# Autodesk Inventor assembly: Computer Case
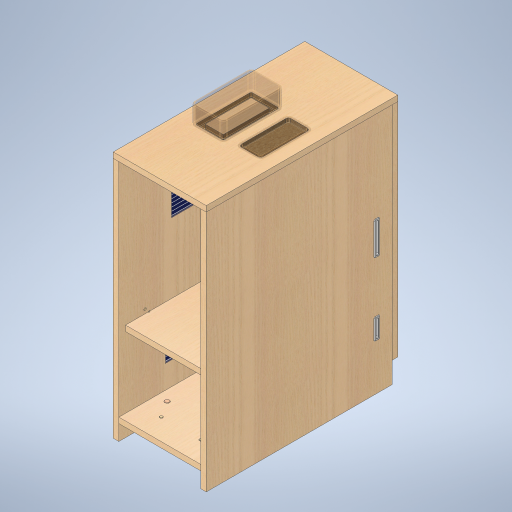
[picture p0: Inventor's stored thumbnail of the model, 512x512]
Saved by Autodesk Inventor 2024 (Build 280153000, 153)
## iProperties
Created: 2023-05-08
Part Number: Computer Case
Document SubType Name: Assembly
Designer: S. Dereškevičius
Author: S. Dereškevičius
## Documents named in this file (21)
- C:\W4INV 2024 Design\PROJECTS\Samples\Macro DEMO\7 Computer Case\Computer Case.iam
- C:\W4INV 2024 Design\PROJECTS\Samples\Macro DEMO\7 Computer Case\CC Right.ipt
- C:\W4INV 2024 Design\PROJECTS\Samples\Macro DEMO\7 Computer Case\CC Top.ipt
- C:\W4INV 2024 Design\PROJECTS\Samples\Macro DEMO\7 Computer Case\CC Left.ipt
- C:\W4INV 2024 Design\PROJECTS\Samples\Macro DEMO\7 Computer Case\CC Bottom.ipt
- C:\W4INV 2024 Design\PROJECTS\Samples\Macro DEMO\7 Computer Case\CC Shelf.ipt
- C:\W4INV 2024 Design\PROJECTS\Samples\Macro DEMO\7 Computer Case\CC Back.ipt
- C:\W4INV 2024 Design\PROJECTS\Samples\Macro DEMO\7 Computer Case\CC Plynth.ipt
- C:\W4INV 2024 Design\PROJECTS\Samples\Macro DEMO\7 Computer Case\Computer Case.iam Smart Hardware\Clamex Joint11\Clamex Joint11.iam
- C:\W4INV 2024 Design\PROJECTS\Samples\Macro DEMO\7 Computer Case\Computer Case.iam Smart Hardware\Clamex Joint12\Clamex Joint12.iam
- C:\W4INV 2024 Design\PROJECTS\Samples\Macro DEMO\7 Computer Case\Computer Case.iam Smart Hardware\Minifix&Dowel Joint 111\Minifix&Dowel Joint 111.iam
- C:\W4INV 2024 Design\PROJECTS\Samples\Macro DEMO\7 Computer Case\Computer Case.iam Smart Hardware\Minifix&Dowel Joint 112\Minifix&Dowel Joint 112.iam
- C:\W4INV 2024 Design\PROJECTS\Samples\Macro DEMO\7 Computer Case\Computer Case.iam Smart Hardware\Shelf Holder Joint11\Shelf Holder Joint11.iam
- C:\W4INV 2024 Design\PROJECTS\Samples\Macro DEMO\7 Computer Case\Computer Case.iam Smart Hardware\Shelf Holder Joint12\Shelf Holder Joint12.iam
- C:\W4INV 2024 Design\PROJECTS\Samples\Macro DEMO\7 Computer Case\Computer Case.iam Smart Hardware\Confirmat Joint11\Confirmat Joint11.iam
- C:\W4INV 2024 Design\PROJECTS\Samples\Macro DEMO\7 Computer Case\Computer Case.iam Smart Hardware\Confirmat Joint12\Confirmat Joint12.iam
- C:\W4INV 2024 Design\PROJECTS\Samples\Macro DEMO\7 Computer Case\Computer Case.iam Smart Hardware\Confirmat Joint14\Confirmat Joint14.iam
- C:\W4INV 2024 Design\PROJECTS\Samples\Macro DEMO\4 Ventilation Grill\Ventilation Grille.ipt
- C:\W4INV 2024 Design\PROJECTS\Samples\Macro DEMO\2 Ways of Macro rotation definition\Table top pencil case.ipt
- C:\W4INV 2024 Design\PROJECTS\Samples\Macro DEMO\3 Alternate Side processing definition\Aisle.ipt
- C:\W4INV 2024 Design\PROJECTS\Samples\Macro DEMO\7 Computer Case\Holder for paper clips-01.ipt
## Components (25 placed, 20 different names)
1. CC Right:1 — Flush:11, Main Plane:1, Main Plane:2
2. CC Top:1 — Flush:1, Align To Edge Plane:3, Table Top:1, Desktop Plane:1, Orientation:1
3. CC Left:1 — Mate:1, Angle:1, Flush:2, Surface for Insertion:1, Surface for Insertion:2
4. CC Bottom:1 — Symmetry:1
5. CC Shelf:1 — Symmetry:1, Flush:9, Main Plane:3
6. CC Back:1 — Surface for Insertion:3, Surface for Insertion:4, Flush:10
7. CC Plynth:1
8. Clamex Joint11:1 [sub-assembly]
9. Clamex Joint12:1 [sub-assembly]
10. Minifix&Dowel Joint 111:1 [sub-assembly]
11. Minifix&Dowel Joint 112:1 [sub-assembly]
12. Shelf Holder Joint11:1 [sub-assembly]
13. Shelf Holder Joint12:1 [sub-assembly]
14. Confirmat Joint11:1 [sub-assembly]
15. Confirmat Joint12:1 [sub-assembly]
16. Confirmat Joint14:1 [sub-assembly]
17. Ventilation Grille:1 — Surface for Insertion:1, Axis Plane 1:1, Axis Plane 2:1, Align To Edge Plane:1
18. Ventilation Grille:2 — Surface for Insertion:2, Axis Plane 1:2, Axis Plane 2:2, Align To Edge Plane:2
19. Ventilation Grille:3 — Surface for Insertion:3, Axis Plane 1:3, Axis Plane 2:3
20. Ventilation Grille:4 — Surface for Insertion:4, Axis Plane 1:4, Axis Plane 2:4, Align To Edge Plane:3
21. Table top pencil case:1 — Table Top:1, Orientation Axis:1, Second Axis:1
22. Aisle:1 — Second Axis:2, Main Plane:1, Orientation Plane:1
23. Aisle:2 — Second Axis:3, Main Plane:2, Orientation Plane:2
24. Aisle:3 — Main Plane:3, Orientation Plane:3, Second Axis:4
25. Holder for paper clips-01:1 — Desktop Plane:1, First Axis:1, Second Axis:5, Orientation:1
## Relationships (39: Mate 19, Flush 14, Angle 5, Symmetry 1)
- Flush:1 (-100 mm): CC Top:1
- Mate:1: CC Left:1
- Angle:1 (0 deg): CC Left:1
- Flush:2 (-580 mm): CC Left:1
- Symmetry:1: CC Bottom:1 ↔ CC Shelf:1
- Surface for Insertion:1 [Flush]: CC Left:1 ↔ Ventilation Grille:1
- Axis Plane 1:1 [Mate]: Ventilation Grille:1
- Axis Plane 2:1 [Mate]: Ventilation Grille:1
- Align To Edge Plane:1 [Angle] (0 deg): Ventilation Grille:1
- Surface for Insertion:2 [Flush]: CC Left:1 ↔ Ventilation Grille:2
- Axis Plane 1:2 [Mate]: Ventilation Grille:2
- Axis Plane 2:2 [Mate]: Ventilation Grille:2
- Align To Edge Plane:2 [Angle] (0 deg): Ventilation Grille:2
- Surface for Insertion:3 [Flush]: CC Back:1 ↔ Ventilation Grille:3
- Axis Plane 1:3 [Mate]: Ventilation Grille:3
- Axis Plane 2:3 [Mate]: Ventilation Grille:3
- Surface for Insertion:4 [Flush]: CC Back:1 ↔ Ventilation Grille:4
- Axis Plane 1:4 [Mate]: Ventilation Grille:4
- Axis Plane 2:4 [Mate]: Ventilation Grille:4
- Align To Edge Plane:3 [Angle] (0 deg): CC Top:1 ↔ Ventilation Grille:4
- Table Top:1 [Flush]: CC Top:1 ↔ Table top pencil case:1
- Orientation Axis:1 [Flush]: Table top pencil case:1
- Second Axis:1 [Mate]: Table top pencil case:1
- Flush:9 (120 mm): CC Shelf:1
- Flush:10 (-80 mm): CC Back:1
- Flush:11 (-50 mm): CC Right:1
- Second Axis:2 [Mate]: Aisle:1
- Main Plane:1 [Mate]: CC Right:1 ↔ Aisle:1
- Orientation Plane:1 [Flush]: Aisle:1
- Second Axis:3 [Mate]: Aisle:2
- Main Plane:2 [Mate]: CC Right:1 ↔ Aisle:2
- Orientation Plane:2 [Flush]: Aisle:2
- Main Plane:3 [Mate]: CC Shelf:1 ↔ Aisle:3
- Orientation Plane:3 [Flush]: Aisle:3
- Second Axis:4 [Mate]: Aisle:3
- Desktop Plane:1 [Mate]: CC Top:1 ↔ Holder for paper clips-01:1
- First Axis:1 [Mate]: Holder for paper clips-01:1
- Second Axis:5 [Mate]: Holder for paper clips-01:1
- Orientation:1 [Angle] (0 deg): CC Top:1 ↔ Holder for paper clips-01:1
